# Autodesk Inventor assembly: commutator_attatchment
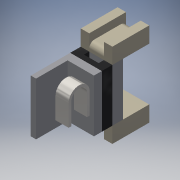
[picture p0: Inventor's stored thumbnail of the model, 180x180]
Saved by Autodesk Inventor 2016 (Build 200138000, 138)
## iProperties
Created: 2016-09-28
Part Number: commutator_attatchment
Document SubType Name: Assembly
Designer: ajar021
Author: ajar021
## Documents named in this file (6)
- C:\Users\ajar021\Documents\CAD files\Commutator_Attachment\commutator_attatchment.iam
- C:\Users\ajar021\Documents\CAD files\Commutator_Attachment\commutator_attachement_front_plate.ipt
- C:\Users\ajar021\Documents\CAD files\Commutator_Attachment\commutator_attachement_side_plate.ipt
- C:\Users\ajar021\Documents\CAD files\Commutator_Attachment\commutator_attachement_cable_cap.ipt
- C:\Users\ajar021\Documents\CAD files\Commutator_Attachment\commutator_attatchment_pulley_bridge.ipt
- E:\band_hook.ipt
## Components (6 placed, 5 different names)
1. commutator_attachement_front_plate:1 — Flush:1, Flush:2, Flush:3, Mate:1, Mate:2
2. commutator_attachement_side_plate:1 — Flush:1, Flush:2
3. commutator_attachement_cable_cap:1 — Flush:3, Flush:4
4. commutator_attatchment_pulley_bridge:1 — Flush:4, Flush:5, Flush:6
5. commutator_attachement_side_plate:2 — Mate:1, Mate:2
6. band_hook:1 — Flush:5, Flush:6
## Relationships (8: Flush 6, Mate 2)
- Flush:1: commutator_attachement_front_plate:1 ↔ commutator_attachement_side_plate:1
- Flush:2: commutator_attachement_front_plate:1 ↔ commutator_attachement_side_plate:1
- Flush:3: commutator_attachement_front_plate:1 ↔ commutator_attachement_cable_cap:1
- Flush:4: commutator_attachement_cable_cap:1 ↔ commutator_attatchment_pulley_bridge:1
- Mate:1: commutator_attachement_front_plate:1 ↔ commutator_attachement_side_plate:2
- Mate:2: commutator_attachement_front_plate:1 ↔ commutator_attachement_side_plate:2
- Flush:5: commutator_attatchment_pulley_bridge:1 ↔ band_hook:1
- Flush:6: commutator_attatchment_pulley_bridge:1 ↔ band_hook:1
